# Autodesk Inventor assembly: Cannon
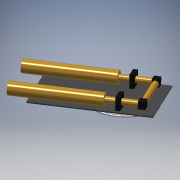
[picture p0: Inventor's stored thumbnail of the model, 180x180]
Saved by Autodesk Inventor 2016 (Build 200138000, 138)
## iProperties
Created: 2018-06-21
Part Number: Cannon
Document SubType Name: Assembly
Designer: Kade
Author: Kade
## Documents named in this file (10)
- F:\Robotics\Off Season\Blannon\Cannon.iam
- F:\Robotics\Off Season\Blannon\Top Plate.ipt
- F:\Robotics\Off Season\Blannon\Turntable.ipt
- F:\Robotics\Off Season\Blannon\Turret Gear.ipt
- F:\Robotics\Off Season\Blannon\Gear and Turntable Connector.ipt
- F:\Robotics\Off Season\Blannon\Cannon Barrel.ipt
- F:\Robotics\Off Season\Blannon\Gear and Barrel Connector.ipt
- F:\Robotics\Off Season\Blannon\Hinge\Working Hinge'.iam
- F:\Robotics\Off Season\Blannon\Cannon Spacer.ipt
- F:\Robotics\Off Season\Blannon\Linear Actuator\Linear Actuator 12inch.iam
## Components (9 placed, 9 different names)
1. Top Plate:1 — Mate:1, Mate:2, Mate:3, Mate:4
2. Turntable:1 — Mate:4, Angle:1, Mate:5, Mate:6, Angle:2, Angle:3, Angle:4, Angle:5
3. Gear and Turntable Connector:1 — Mate:6, Angle:2, Mate:7, Mate:8
4. Turret Gear:1 — Mate:8, Mate:9, Angle:3, Mate:11, Mate:13, Mate:14
5. Gear and Barrel Connector:1 — Mate:10, Angle:4, Mate:11, Mate:12
6. Cannon Spacer:1 — Mate:12, Angle:5, Mate:13, Mate:14, Mate:15, Flush:1, Flush:2, Flush:4
7. Working Hinge':1 [sub-assembly] — Mate:15, Flush:1, Flush:2, Mate:16, Flush:3
8. Cannon Barrel:1 — Mate:16, Flush:3, Flush:4
9. Linear Actuator 12inch:1 [sub-assembly]
## Relationships (25: Mate 16, Angle 5, Flush 4)
- Mate:1: Top Plate:1
- Mate:2: Top Plate:1
- Mate:3: Top Plate:1
- Mate:4: Top Plate:1 ↔ Turntable:1
- Angle:1 (-120 deg): Turntable:1
- Mate:5: Turntable:1
- Mate:6: Turntable:1 ↔ Gear and Turntable Connector:1
- Angle:2 (0 deg): Turntable:1 ↔ Gear and Turntable Connector:1
- Mate:7: Gear and Turntable Connector:1
- Mate:8: Gear and Turntable Connector:1 ↔ Turret Gear:1
- Mate:9: Turret Gear:1
- Angle:3 (0 deg): Turntable:1 ↔ Turret Gear:1
- Mate:10: Gear and Barrel Connector:1
- Angle:4 (0 deg): Turntable:1 ↔ Gear and Barrel Connector:1
- Mate:11: Turret Gear:1 ↔ Gear and Barrel Connector:1
- Mate:12: Gear and Barrel Connector:1 ↔ Cannon Spacer:1
- Angle:5 (0 deg): Turntable:1 ↔ Cannon Spacer:1
- Mate:13 (-152.4 mm): Turret Gear:1 ↔ Cannon Spacer:1
- Mate:14 (-42.0751 mm): Turret Gear:1 ↔ Cannon Spacer:1
- Mate:15: Cannon Spacer:1 ↔ Working Hinge':1
- Flush:1: Cannon Spacer:1 ↔ Working Hinge':1
- Flush:2 (12.7 mm): Cannon Spacer:1 ↔ Working Hinge':1
- Mate:16: Working Hinge':1 ↔ Cannon Barrel:1
- Flush:3 (-508 mm): Working Hinge':1 ↔ Cannon Barrel:1
- Flush:4 (-110.3249 mm): Cannon Spacer:1 ↔ Cannon Barrel:1
